# Autodesk Inventor assembly: TiltMount
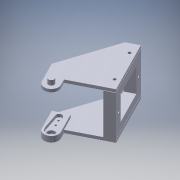
[picture p0: Inventor's stored thumbnail of the model, 180x180]
Saved by Autodesk Inventor 2017 (Build 210142000, 142)
## iProperties
Created: 2017-03-10
Part Number: TiltMount
Document SubType Name: Assembly
Designer: Naga
Author: Naga
## Documents named in this file (4)
- E:\GDrive\IEEE CS\SoutheastCon2017\Cad\tilt\TiltMount.iam
- E:\GDrive\IEEE CS\SoutheastCon2017\Cad\tilt\bottomTiltOnly.ipt
- E:\GDrive\IEEE CS\SoutheastCon2017\Cad\tilt\servoSide_std.ipt
- E:\GDrive\IEEE CS\SoutheastCon2017\Cad\tilt\sideShaft.ipt
## Components (3 placed, 3 different names)
1. bottomTiltOnly:1 — Mate:3, Mate:4, Mate:5, Mate:6, Mate:7, Mate:8
2. sideShaft:1 — Mate:5, Mate:6, Mate:8
3. servoSide_std:1 — Mate:3, Mate:4, Mate:7
## Relationships (6: Mate 6)
- Mate:3: bottomTiltOnly:1 ↔ servoSide_std:1
- Mate:4: bottomTiltOnly:1 ↔ servoSide_std:1
- Mate:5: bottomTiltOnly:1 ↔ sideShaft:1
- Mate:6: bottomTiltOnly:1 ↔ sideShaft:1
- Mate:7: bottomTiltOnly:1 ↔ servoSide_std:1
- Mate:8: bottomTiltOnly:1 ↔ sideShaft:1
